# Autodesk Inventor assembly: RewindingSpoolAssembly
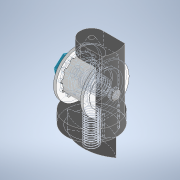
[picture p0: Inventor's stored thumbnail of the model, 180x180]
Saved by Autodesk Inventor 2021 (Build 250183000, 183)
## iProperties
Created: 2020-10-05
Part Number: RewindingSpoolAssembly
Document SubType Name: Assembly
Designer: elmar
Author: elmar
## Documents named in this file (9)
- D:\FourWireBraidingMachine\InventorFiles\RewindingSpoolAssembly.iam
- D:\FourWireBraidingMachine\InventorFiles\RewindingSpoolHolder.ipt
- D:\FourWireBraidingMachine\InventorFiles\RewingingSpoolBushing.ipt
- D:\FourWireBraidingMachine\InventorFiles\RewindingSpool.ipt
- D:\FourWireBraidingMachine\InventorFiles\Spring.ipt
- D:\FourWireBraidingMachine\InventorFiles\SpoolClutchFixedPlate.ipt
- C:\Users\elmar\OneDrive\Documents\Inventor\Content Center Files\R2021\en-US\GB_T 5782-2000\Bolt GB_T 5782 M3 x 30.ipt
- C:\Users\elmar\OneDrive\Documents\Inventor\Content Center Files\R2021\en-US\AS 1237 (2.1)\AS 1237 - 3.ipt
- C:\Users\elmar\OneDrive\Documents\Inventor\Content Center Files\R2021\en-US\AS 1112 (2)\AS 1112 - M3  Type 5.ipt
## Components (8 placed, 8 different names)
1. RewindingSpoolHolder:1 — Insert:1, Insert:2, Angle:2
2. RewingingSpoolBushing:1 — Mate:2, Insert:4, Mate:4
3. RewindingSpool:1 — Insert:3, Mate:3
4. Spring:1 — Mate:1, Mate:3, Mate:4
5. SpoolClutchFixedPlate:1 — Insert:4, Insert:5, Angle:1
6. Bolt GB/T 5782-2000 M3x30:1 — Insert:1, Mate:1, Mate:2, Angle:2
7. AS 1237 (2.1) 3:1 — Insert:2, Insert:3
8. AS 1112 (2) - Metric M3  Type 5:1 — Insert:5, Angle:1
## Relationships (11: Insert 5, Mate 4, Angle 2)
- Insert:1: RewindingSpoolHolder:1 ↔ Bolt GB/T 5782-2000 M3x30:1
- Insert:2: RewindingSpoolHolder:1 ↔ AS 1237 (2.1) 3:1
- Insert:3: RewindingSpool:1 ↔ AS 1237 (2.1) 3:1
- Mate:1: Spring:1 ↔ Bolt GB/T 5782-2000 M3x30:1
- Mate:2: RewingingSpoolBushing:1 ↔ Bolt GB/T 5782-2000 M3x30:1
- Insert:4: RewingingSpoolBushing:1 ↔ SpoolClutchFixedPlate:1
- Insert:5: SpoolClutchFixedPlate:1 ↔ AS 1112 (2) - Metric M3  Type 5:1
- Angle:1 (0 deg): SpoolClutchFixedPlate:1 ↔ AS 1112 (2) - Metric M3  Type 5:1
- Angle:2 (0 deg): RewindingSpoolHolder:1 ↔ Bolt GB/T 5782-2000 M3x30:1
- Mate:3: RewindingSpool:1 ↔ Spring:1
- Mate:4: RewingingSpoolBushing:1 ↔ Spring:1
